# Autodesk Inventor assembly: HipJoint_MIR
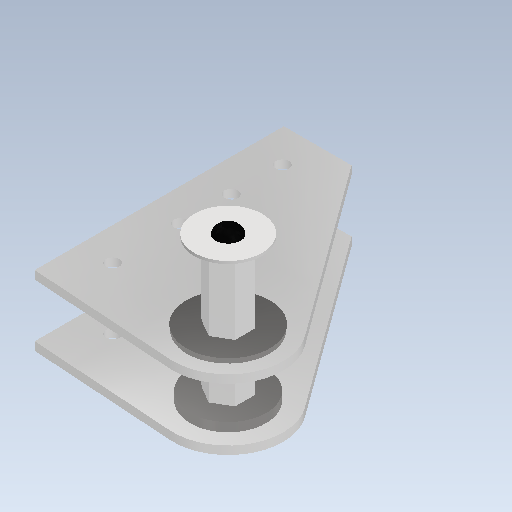
[picture p0: Inventor's stored thumbnail of the model, 512x512]
Saved by Autodesk Inventor 2023 (Build 270158000, 158)
## iProperties
Created: 2023-02-11
Part Number: HipJoint_MIR
Document SubType Name: Assembly
Designer: Dave
Author: coled
## Documents named in this file (6)
- C:\Users\Dave\Documents\GitHub\BehrendURCMechanical\CAD\Chassis\HipJoint_MIR.iam
- C:\Users\Dave\Documents\GitHub\BehrendURCMechanical\CAD\Chassis\Bearing_MIR.ipt
- C:\Users\Dave\Documents\GitHub\BehrendURCMechanical\CAD\Chassis\Bracket_MIR.ipt
- C:\Users\Dave\Documents\GitHub\BehrendURCMechanical\CAD\Chassis\HexShaft_MIR.ipt
- C:\Users\Dave\Documents\GitHub\BehrendURCMechanical\CAD\Chassis\Washer_MIR.ipt
- C:\Users\Dave\Documents\GitHub\BehrendURCMechanical\CAD\Chassis\Screw_MIR.ipt
## Components (9 placed, 5 different names)
1. Bearing_MIR:1 — Mate:2, Mate:1, Mate:4
2. Bracket_MIR:1 — Mate:2, Mate:1, Mate:3
3. Bracket_MIR:2 — Mate:4, Mate:3, Mate:6, Mate:5
4. Bearing_MIR:2 — Mate:6, Mate:5, Flush:1, Mate:7, Mate:8
5. HexShaft_MIR:1 — Flush:1, Mate:7, Mate:11, Mate:10, Mate:9, Mate:16
6. Washer_MIR:1 — Mate:11, Mate:10, Mate:15, Mate:14
7. Washer_MIR:2 — Mate:9, Mate:8, Mate:12
8. Screw_MIR:1 — Mate:15, Mate:14
9. Screw_MIR:2 — Mate:16, Mate:12
## Relationships (16: Mate 15, Flush 1)
- Mate:2: Bearing_MIR:1 ↔ Bracket_MIR:1
- Mate:1: Bearing_MIR:1 ↔ Bracket_MIR:1
- Mate:4: Bearing_MIR:1 ↔ Bracket_MIR:2
- Mate:3 (20 mm): Bracket_MIR:1 ↔ Bracket_MIR:2
- Mate:6: Bracket_MIR:2 ↔ Bearing_MIR:2
- Mate:5: Bracket_MIR:2 ↔ Bearing_MIR:2
- Flush:1: Bearing_MIR:2 ↔ HexShaft_MIR:1
- Mate:7: Bearing_MIR:2 ↔ HexShaft_MIR:1
- Mate:11: HexShaft_MIR:1 ↔ Washer_MIR:1
- Mate:10: HexShaft_MIR:1 ↔ Washer_MIR:1
- Mate:9: HexShaft_MIR:1 ↔ Washer_MIR:2
- Mate:8: Bearing_MIR:2 ↔ Washer_MIR:2
- Mate:15: Washer_MIR:1 ↔ Screw_MIR:1
- Mate:14: Washer_MIR:1 ↔ Screw_MIR:1
- Mate:16: HexShaft_MIR:1 ↔ Screw_MIR:2
- Mate:12: Washer_MIR:2 ↔ Screw_MIR:2
